# Autodesk Inventor assembly: tube
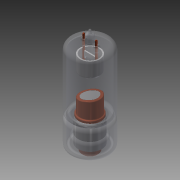
[picture p0: Inventor's stored thumbnail of the model, 180x180]
Saved by Autodesk Inventor 2015 (Build 190159000, 159)
## iProperties
Created: 2014-09-24
Part Number: tube
Document SubType Name: Assembly
Designer: Adam
Author: Adam
## Documents named in this file (6)
- C:\Users\Adam\Desktop\xray_1\tube.iam
- C:\Users\Adam\Desktop\xray_1\tube.ipt
- C:\Users\Adam\Desktop\xray_1\anode-bell.ipt
- C:\Users\Adam\Desktop\xray_1\anode-copper.ipt
- C:\Users\Adam\Desktop\xray_1\tungsten.ipt
- C:\Users\Adam\Desktop\xray_1\cathode-ring-1.ipt
## Components (5 placed, 5 different names)
1. tube:1 — Flush:1, Flush:5
2. anode-bell:1 — Flush:1, Flush:2
3. anode-copper:1 — Flush:2, Flush:3, Flush:4
4. tungsten:1 — Flush:3, Flush:4
5. cathode-ring-1:1 — Flush:5
## Relationships (5: Flush 5)
- Flush:1: tube:1 ↔ anode-bell:1
- Flush:2: anode-bell:1 ↔ anode-copper:1
- Flush:3: anode-copper:1 ↔ tungsten:1
- Flush:4: anode-copper:1 ↔ tungsten:1
- Flush:5: tube:1 ↔ cathode-ring-1:1
